# Autodesk Inventor assembly: lados
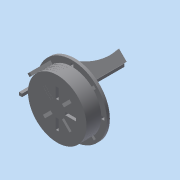
[picture p0: Inventor's stored thumbnail of the model, 180x180]
Saved by Autodesk Inventor 2015 (Build 190159000, 159)
## iProperties
Created: 2017-10-02
Part Number: lados
Document SubType Name: Assembly
Designer: macbook
Author: macbook
## Documents named in this file (4)
- \\Mac\Home\Dropbox\cosplay\espalda\lados\lados.iam
- \\Mac\Home\Dropbox\cosplay\espalda\lados\base.ipt
- \\Mac\Home\Dropbox\cosplay\espalda\lados\brazos.ipt
- \\Mac\Home\Dropbox\cosplay\espalda\lados\medio.ipt
## Components (8 placed, 3 different names)
1. base:1 — Mate:1, Mate:2, Mate:3, Rigid:3, Mate:4, Mate:5, Mate:6
2. brazos:1 — Mate:4, Mate:5, Mate:6
3. brazos:2 — Mate:1, Mate:2, Mate:3
4. medio:1 — Rigid:2, Rigid:3
5. medio:2 — Rigid:1, Rigid:2
6. medio:3 — Rigid:1, Rotational:1
7. medio:4 — Rotational:1, Rigid:4
8. medio:5 — Rigid:4
## Relationships (11: Mate 6, WeldJoint 4, RevoluteJoint 1)
- Mate:1: base:1 ↔ brazos:2
- Mate:2: base:1 ↔ brazos:2
- Mate:3: base:1 ↔ brazos:2
- Rigid:1 [WeldJoint]: medio:2 ↔ medio:3
- Rigid:2 [WeldJoint]: medio:1 ↔ medio:2
- Rigid:3 [WeldJoint]: base:1 ↔ medio:1
- Rotational:1 [RevoluteJoint]: medio:3 ↔ medio:4
- Rigid:4 [WeldJoint]: medio:4 ↔ medio:5
- Mate:4: base:1 ↔ brazos:1
- Mate:5: base:1 ↔ brazos:1
- Mate:6: base:1 ↔ brazos:1
